# Autodesk Inventor assembly: Tiger
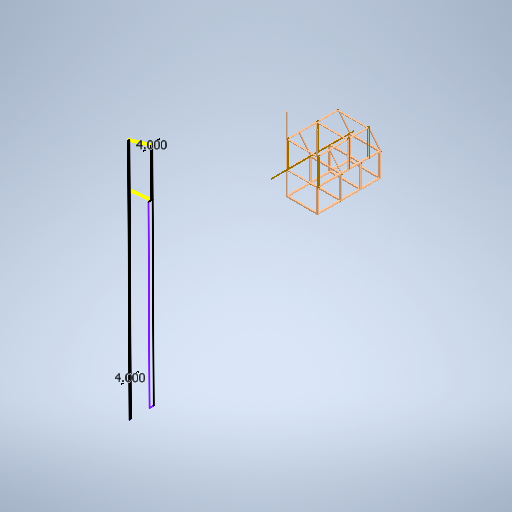
[picture p0: Inventor's stored thumbnail of the model, 512x512]
Saved by Autodesk Inventor 2025 (Build 290162000, 162)
## iProperties
Created: 2024-06-05
Part Number: Tiger
Document SubType Name: Assembly
Designer: Cupri
Mass: 180546 g
Surface Area: 136258 cm^2
Volume: 328266 cm^3
Density: 0.55 g/cm^3
Author: Cupri
## Documents named in this file (44)
- C:\Users\Win\Documents\GitHub\USCTigerBurn24\v2\Tiger.iam
- C:\Users\Win\Documents\GitHub\USCTigerBurn24\Standard Timber\4x4x72.ipt
- C:\Users\Win\Documents\GitHub\USCTigerBurn24\Standard Timber\4x4x40.ipt
- C:\Users\Win\Documents\GitHub\USCTigerBurn24\Standard Timber\2x4x36.ipt
- C:\Users\Win\Documents\GitHub\USCTigerBurn24\Standard Timber\2x4x40.ipt
- C:\Users\Win\Documents\GitHub\USCTigerBurn24\Standard Timber\2x4x24.ipt
- C:\Users\Win\Documents\GitHub\USCTigerBurn24\Standard Timber\2x4x28.ipt
- C:\Users\Win\Documents\GitHub\USCTigerBurn24\Standard Timber\2x4x72 (45 90).ipt
- C:\Users\Win\Documents\GitHub\USCTigerBurn24\Standard Timber\2x4x68 (45 90).ipt
- C:\Users\Win\Documents\GitHub\USCTigerBurn24\Standard Timber\2x4x42.343 (45 90).ipt
- C:\Users\Win\Documents\GitHub\USCTigerBurn24\Standard Timber\2x4x72 (30 90).ipt
- C:\Users\Win\Documents\GitHub\USCTigerBurn24\Standard Timber\2x4x44.ipt
- C:\Users\Win\Documents\GitHub\USCTigerBurn24\Standard Timber\4x4x104.303.ipt
- C:\Users\Win\Documents\GitHub\USCTigerBurn24\Standard Timber\4x4xigiveup.ipt
- C:\Users\Win\Documents\GitHub\USCTigerBurn24\Standard Timber\4x4x96.ipt
- C:\Users\Win\Documents\GitHub\USCTigerBurn24\Standard Timber\2x4x96.ipt
- C:\Users\Win\Documents\GitHub\USCTigerBurn24\Standard Timber\2x4xidk.ipt
- C:\Users\Win\Documents\GitHub\USCTigerBurn24\Standard Timber\2x4x120.ipt
- C:\Users\Win\Documents\GitHub\USCTigerBurn24\Standard Timber\2x4x72.ipt
- C:\Users\Win\Documents\GitHub\USCTigerBurn24\Standard Timber\2x4x88.ipt
- C:\Users\Win\Documents\GitHub\USCTigerBurn24\Standard Timber\4x4x55.ipt
- C:\Users\Win\Documents\GitHub\USCTigerBurn24\Standard Timber\4x4x66.ipt
- C:\Users\Win\Documents\GitHub\USCTigerBurn24\Standard Timber\2x4x48.ipt
- C:\Users\Win\Documents\GitHub\USCTigerBurn24\Standard Timber\leg slant.ipt
- C:\Users\Win\Documents\GitHub\USCTigerBurn24\Standard Timber\Leg slant.2.ipt
- C:\Users\Win\Documents\GitHub\USCTigerBurn24\Standard Timber\2x4x48_MIR.ipt
- C:\Users\Win\Documents\GitHub\USCTigerBurn24\Standard Timber\2x4x72_MIR.ipt
- C:\Users\Win\Documents\GitHub\USCTigerBurn24\Standard Timber\2x4x36_MIR.ipt
- C:\Users\Win\Documents\GitHub\USCTigerBurn24\Standard Timber\2x4x24_MIR.ipt
- C:\Users\Win\Documents\GitHub\USCTigerBurn24\Standard Timber\2x4x28_MIR.ipt
- C:\Users\Win\Documents\GitHub\USCTigerBurn24\Standard Timber\leg slant_MIR.ipt
- C:\Users\Win\Documents\GitHub\USCTigerBurn24\Standard Timber\Leg slant.2_MIR.ipt
- C:\Users\Win\Documents\GitHub\USCTigerBurn24\Standard Timber\back slant.ipt
- C:\Users\Win\Documents\2x4x76.ipt
- C:\Users\Win\Documents\2X4X65.191.ipt
- C:\Users\Win\Documents\2X4X92.ipt
- C:\Users\Win\Documents\wrapping paper.ipt
- C:\Users\Win\Documents\paperbodyfront.ipt
- C:\Users\Win\Documents\GitHub\USCTigerBurn24\v2\Tiger\AIP\FEA\epzzwi8io.fins
- C:\Users\Win\Documents\GitHub\USCTigerBurn24\v2\Tiger\AIP\FEA\epzzwi8io.fsat
- C:\Users\Win\Documents\GitHub\USCTigerBurn24\v2\Tiger\AIP\FEA\epzzwi8io.ftes
- C:\Users\Win\Documents\GitHub\USCTigerBurn24\v2\Tiger\AIP\FEA\epzzwi8io.fwiz
- C:\Users\Win\Documents\GitHub\USCTigerBurn24\v2\Tiger\AIP\FEA\epzzwi8jk.fmsh
- C:\Users\Win\Documents\GitHub\USCTigerBurn24\v2\Tiger\AIP\FEA\epzzwi8jl.fres
## Components (212 placed, 37 different names)
1. 4x4x104.303:1 — Flush:221, Flush:222
2. 4x4x104.303:2 — Flush:221, Flush:222
3. 4x4xigiveup:1 — Mate:186
4. 4x4xigiveup:2 — Flush:237, Mate:187, Mate:188
5. 4x4x96:1 — Flush:232
6. 4x4x96:2 — Flush:232
7. 4x4x96:3 — Flush:230
8. 4x4x96:4 — Flush:230
9. 4x4x96:5
10. 2x4x96:1 — Mate:186, Flush:237, Mate:187, Mate:188, Mate:191
11. 2x4xidk:1 — Mate:189, Mate:190, Mate:191, Flush:241
12. 2x4xidk:2 — Mate:192, Flush:240, Flush:241
13. 4x4x66:3 — Mate:391, Flush:531, Flush:532, Mate:401
14. 4x4x66:4 — Mate:392, Flush:533, Flush:534, Flush:548, Mate:402
15. 4x4x66:5 — Mate:393, Flush:535, Flush:536, Flush:606
16. 4x4x66:6 — Flush:537, Mate:394, Flush:538
17. 4x4x66:7 — Mate:395, Flush:539, Flush:540, Mate:403
18. 4x4x66:8 — Mate:396, Flush:541, Flush:542, Flush:563
19. 4x4x66:9 — Mate:397, Flush:543, Flush:544
20. 4x4x66:10 — Mate:398, Flush:545, Flush:546, Mate:399, Flush:547
21. 2x4x120:6 — Flush:561, Flush:565, Flush:566, Flush:567, Mate:419, Flush:572, Mate:431, Flush:584
22. 2x4x120:7 — Flush:563, Flush:564, Mate:415, Mate:416, Flush:568, Mate:417, Mate:433, Flush:585
23. 2x4x72:11 — Mate:414, Flush:571, Mate:430, Flush:582, Flush:583
24. 2x4x72:12 — Flush:580, Flush:581, Mate:429
25. 2x4x88:5 — Mate:413, Flush:562
26. 2x4x88:6 — Flush:569
27. 2x4x88:7 — Flush:570, Mate:418, Mate:420, Flush:606
28. back slant:1 — Flush:565, Flush:566, Flush:567, Mate:437, Mate:438, Flush:588
29. back slant:2 — Mate:415, Mate:416, Flush:568, Mate:435, Mate:436, Flush:586
30. back slant:3 — Mate:417, Flush:571, Mate:418
31. back slant:4 — Mate:419, Flush:572, Mate:420, Flush:598, Flush:599
32. 2x4x76:5 — Flush:580, Flush:581, Mate:429, Mate:432, Flush:589, Flush:590, Flush:607
33. 2x4x76:6 — Mate:430, Flush:582, Flush:583, Mate:434, Flush:591, Mate:439, Flush:592
34. 2X4X65.191:3 — Mate:435, Mate:436, Flush:586, Flush:587, Mate:442, Flush:597, Mate:443
35. 2X4X65.191:4 — Mate:437, Mate:438, Flush:588, Flush:595
36. 2x4x76:7 — Mate:431, Flush:584, Mate:432, Flush:596
37. 2x4x76:8 — Mate:433, Flush:585, Mate:434, Flush:587
38. 2X4X92:1 — Flush:589, Flush:590, Mate:440, Flush:593, Flush:594, Mate:441, Mate:444, Flush:602, Flush:603, Flush:607
39. 2X4X92:2 — Flush:591, Mate:439, Flush:592, Mate:445, Flush:604, Flush:605
40. 2x4x88:9 — Mate:440, Flush:593, Flush:594, Flush:600
41. 2x4x88:10 — Mate:441, Flush:595, Flush:596
42. 2X4X92:3 — Mate:442, Flush:597, Mate:443
43. wrapping paper:1 — Flush:598, Flush:599
44. paperbodyfront:1 — Flush:600, Flush:601
45. 2x4x72:13 — Mate:445, Flush:604, Flush:605
46. 2x4x72:15 — Mate:444, Flush:602, Flush:603
47. 2x4x72 (45 90):1 — Flush:88
48. 2x4x68 (45 90):1 — Flush:44, Flush:88
49. 2x4x72 (45 90):2 — Flush:48, Mate:48, Flush:51, Mate:49
50. 2x4x72 (45 90):3 — Flush:44, Mate:45, Mate:50, Flush:52, Mate:51
51. 2x4x42.343 (45 90):1 — Flush:48
52. 2x4x42.343 (45 90):2 — Mate:45
53. 2x4x72 (30 90):1 — Mate:48, Flush:51, Mate:49, Flush:70, Flush:238, Mate:192, Flush:240
54. 2x4x72 (30 90):2 — Mate:50, Flush:52, Mate:51, Flush:71, Flush:72
55. 2x4x72 (45 90):4 — Mate:61, Flush:61, Flush:62
56. 2x4x68 (45 90):2 — Mate:61, Flush:61, Flush:62
57. 2x4x72 (45 90):5 — Flush:59, Mate:59, Mate:65, Flush:67, Flush:68
58. 2x4x72 (45 90):6 — Flush:63, Flush:64, Mate:68, Flush:73
59. 2x4x42.343 (45 90):3 — Flush:59, Mate:59
60. 2x4x42.343 (45 90):4 — Flush:63
61. 2x4x72 (30 90):3 — Mate:66, Flush:69, Flush:204, Mate:189
62. 2x4x72 (30 90):4 — Flush:64, Mate:67, Mate:69, Flush:239
63. 2x4x44:1 — Mate:67, Flush:71, Flush:72, Flush:239, Mate:190
64. 2x4x44:2 — Mate:65, Flush:67, Flush:68
65. 2x4x44:3 — Mate:66, Flush:69, Flush:70, Flush:204, Flush:238
66. 2x4x44:4 — Mate:68, Flush:73, Mate:69
67. 4x4x72:65
68. 4x4x72:66
69. 4x4x40:117
70. 4x4x40:118
71. 4x4x40:119
72. 4x4x40:120
73. 4x4x40:121
74. 4x4x40:122
75. 4x4x40:123
76. 4x4x40:124
77. 4x4x72:67
78. 4x4x72:68
79. 4x4x40:125
80. 4x4x40:126
81. 4x4x40:127
82. 2x4x40:7
83. 2x4x36:25
84. 2x4x36:26
85. 2x4x36:27
86. 2x4x36:28
87. 2x4x24:13
88. 2x4x24:14
89. 2x4x28:13
90. 2x4x28:14
91. 4x4x72:69
92. 4x4x72:70
93. 4x4x40:128
94. 4x4x40:129
95. 4x4x40:130
96. 4x4x40:131
97. 4x4x72:71
98. 4x4x72:72
99. 4x4x72:73
100. 4x4x72:74
101. 4x4x40:132
102. 4x4x40:133
103. 4x4x40:134
104. 4x4x40:135
105. 4x4x40:136
106. 4x4x40:137
107. 4x4x40:138
108. 4x4x40:139
109. 4x4x72:75
110. 4x4x72:76
111. 4x4x40:140
112. 4x4x40:141
113. 4x4x40:142
114. 2x4x40:8
115. 2x4x36:29
116. 2x4x36:30
117. 2x4x36:31
118. 2x4x36:32
119. 2x4x24:15
120. 2x4x24:16
121. 2x4x28:15
122. 2x4x28:16
123. 4x4x72:77
124. 4x4x72:78
125. 4x4x40:143
126. 4x4x40:144
127. 4x4x40:145
128. 4x4x40:146
129. 4x4x72:79
130. 4x4x72:80
131. 4x4x96:7 — Flush:393, Mate:316, Flush:405, Mate:318, Mate:393, Flush:535, Flush:536, Mate:398, Flush:545, Flush:546
132. 4x4x96:10 — Flush:396, Mate:314, Flush:397, Flush:399, Mate:395, Flush:539, Flush:540, Mate:396, Flush:541, Flush:542
133. 2x4x120:4 — Mate:303, Flush:371, Flush:372, Flush:385, Mate:310, Flush:386, Flush:387, Mate:311, Flush:389, Mate:312, Mate:403, Flush:561
134. 2x4x120:5 — Mate:302, Flush:369, Flush:370, Mate:414, Flush:564
135. 2x4x72:1 — Mate:302, Flush:369, Flush:370, Mate:399, Flush:547, Flush:548, Mate:400, Mate:402
136. 2x4x72:2 — Mate:303, Flush:371, Flush:372, Flush:391, Mate:313, Flush:549, Mate:401
137. 4x4x96:13 — Flush:403, Flush:404, Flush:406, Mate:317, Mate:391, Flush:531, Flush:532, Mate:392, Flush:533, Flush:534
138. 4x4x96:16 — Flush:394, Flush:395, Mate:315, Flush:400, Flush:401, Flush:537, Mate:394, Flush:538, Mate:397, Flush:543, Flush:544
139. 2x4x88:1 — Flush:385, Mate:310, Flush:386, Mate:413, Flush:562
140. 2x4x88:2 — Flush:387, Mate:311, Flush:569
141. 2x4x88:3 — Flush:389, Mate:312, Flush:570, Flush:601
142. 2x4x88:4 — Flush:391, Mate:313, Mate:400, Flush:549
143. 4x4x55:1 — Flush:393, Flush:394, Flush:395
144. 4x4x55:2 — Flush:396, Mate:314, Flush:397, Flush:527
145. 4x4x55:3 — Flush:399, Mate:315, Flush:530
146. 4x4x55:4 — Flush:400, Mate:316, Flush:401, Mate:389
147. 4x4x66:1 — Flush:403, Flush:404, Mate:318
148. 4x4x66:2 — Flush:405, Flush:406, Mate:317
149. 2x4x48:1 — Mate:319, Flush:407, Flush:408, Mate:322, Mate:330, Flush:422, Flush:423
150. 2x4x48:2 — Flush:409, Mate:320, Flush:410, Mate:321, Flush:411, Mate:328, Flush:419, Flush:461, Mate:347, Flush:527
151. 2x4x48:3 — Mate:319, Flush:407, Flush:408, Flush:409, Mate:320, Flush:410, Mate:327, Flush:417, Flush:418
152. 2x4x48:4 — Mate:321, Flush:411, Mate:322, Mate:329, Flush:420, Flush:421
153. 2x4x48:5 — Flush:452
154. 2x4x48:6 — Flush:426, Flush:427
155. 2x4x48:7 — Mate:331, Flush:424, Flush:425, Flush:430, Flush:431, Flush:453, Mate:339
156. 2x4x48:8 — Flush:428, Flush:429
157. 2x4x72:3 — Mate:327, Flush:417, Flush:418, Mate:331, Flush:424, Flush:425, Flush:430, Flush:431
158. 2x4x72:4 — Mate:328, Flush:419, Flush:426, Flush:427, Mate:346, Flush:462
159. 2x4x72:5 — Mate:329, Flush:420, Flush:421, Flush:428, Flush:429, Flush:464
160. 2x4x72:6 — Mate:330, Flush:422, Flush:423
161. 2x4x48:9 — Flush:445, Flush:446
162. 2x4x48:10 — Mate:337, Flush:449, Flush:450
163. 2x4x48:11
164. 2x4x48:12 — Flush:447, Flush:448, Mate:338, Mate:349, Flush:465, Flush:466
165. 2x4x72:7 — Flush:452, Flush:453, Mate:339
166. 2x4x72:8 — Mate:337, Flush:449, Flush:450
167. 2x4x72:9 — Flush:447, Flush:448, Flush:451, Mate:338
168. 2x4x72:10 — Flush:445, Flush:446, Flush:451
169. 2x4x36:33
170. 2x4x36:34 — Flush:463, Flush:464
171. 2x4x36:35 — Mate:348, Mate:390
172. 2x4x36:36 — Flush:461, Mate:347
173. 2x4x24:17
174. 2x4x24:18 — Mate:390
175. 2x4x28:17
176. 2x4x28:18
177. 2x4x48:13 — Mate:346, Flush:462, Mate:348, Flush:463
178. 2x4x48:14 — Mate:349, Flush:465, Flush:466, Flush:467, Flush:468, Flush:469, Flush:470
179. leg slant:1 — Flush:467, Flush:468
180. Leg slant.2:1 — Flush:469, Flush:470
181. 2x4x48_MIR:1 — Flush:473, Flush:474, Mate:351, Mate:352, Flush:494, Flush:495, Mate:362
182. 2x4x48_MIR:2 — Flush:471, Mate:350, Flush:472, Flush:475, Mate:353, Flush:489, Mate:360, Mate:371, Flush:519
183. 2x4x48_MIR:3 — Flush:471, Mate:350, Flush:472, Flush:473, Flush:474, Mate:351, Flush:485, Flush:486, Mate:359
184. 2x4x48_MIR:4 — Mate:352, Flush:475, Mate:353, Flush:492, Flush:493, Mate:361, Flush:530
185. 2x4x48_MIR:5 — Flush:477, Flush:479, Mate:355, Mate:356, Flush:502
186. 2x4x48_MIR:6 — Mate:354, Flush:476, Flush:478, Flush:480, Mate:357, Flush:487, Flush:488
187. 2x4x48_MIR:7 — Mate:354, Flush:476, Flush:477, Flush:478, Flush:479, Mate:355, Flush:481, Flush:482, Flush:483, Flush:484, Mate:358, Mate:367, Flush:501
188. 2x4x48_MIR:8 — Mate:356, Flush:480, Mate:357, Flush:490, Flush:491
189. 2x4x72_MIR:1 — Flush:481, Flush:482, Flush:483, Flush:484, Mate:358, Flush:485, Flush:486, Mate:359
190. 2x4x72_MIR:2 — Flush:487, Flush:488, Flush:489, Mate:360, Flush:524, Mate:377
191. 2x4x72_MIR:3 — Flush:490, Flush:491, Flush:492, Flush:493, Mate:361, Flush:518, Mate:389
192. 2x4x72_MIR:4 — Flush:494, Flush:495, Mate:362
193. 2x4x48_MIR:9 — Flush:497, Flush:499, Mate:364, Mate:365, Flush:516, Flush:517, Mate:385, Mate:404
194. 2x4x48_MIR:10 — Mate:363, Flush:496, Flush:498, Flush:500, Mate:366, Flush:507, Flush:508, Mate:369, Flush:509, Flush:510, Flush:529, Mate:387
195. 2x4x48_MIR:11 — Mate:363, Flush:496, Flush:497, Flush:498, Flush:499, Mate:364, Flush:503, Flush:504, Flush:505, Mate:368, Flush:506
196. 2x4x48_MIR:12 — Mate:365, Flush:500, Mate:366, Mate:370, Flush:511, Flush:512, Flush:513, Flush:514, Flush:525, Flush:526, Mate:378
197. 2x4x72_MIR:5 — Mate:367, Flush:501, Flush:502, Flush:503, Flush:504, Flush:505, Mate:368, Flush:506
198. 2x4x72_MIR:6 — Flush:507, Flush:508, Mate:369, Flush:509, Flush:510
199. 2x4x72_MIR:7 — Mate:370, Flush:511, Flush:512, Flush:513, Flush:514, Flush:515
200. 2x4x72_MIR:8 — Flush:515, Flush:516, Flush:517
201. 2x4x36_MIR:1 — Flush:522, Mate:375, Rigid:233
202. 2x4x36_MIR:2 — Flush:518, Mate:373, Flush:520, Mate:374, Flush:521, Flush:523
203. 2x4x36_MIR:3 — Mate:372, Mate:376, Rigid:235, Mate:388
204. 2x4x36_MIR:4 — Mate:371, Flush:519, Mate:372, Rigid:234, Rigid:236
205. 2x4x24_MIR:1 — Mate:373, Flush:520, Rigid:233
206. 2x4x24_MIR:2 — Rigid:234, Mate:388
207. 2x4x28_MIR:1 — Mate:374, Flush:521, Rigid:235
208. 2x4x28_MIR:2 — Flush:522, Mate:375, Rigid:236
209. 2x4x48_MIR:13 — Flush:523, Mate:376, Flush:524, Mate:377
210. 2x4x48_MIR:14 — Flush:525, Flush:526, Mate:378, Mate:379, Mate:380, Mate:381, Mate:382, Mate:384, Mate:386, Flush:550, Mate:405
211. leg slant_MIR:1 — Mate:379, Mate:380, Mate:384, Mate:385, Mate:404, Flush:550, Mate:405
212. Leg slant.2_MIR:1 — Mate:381, Mate:382, Mate:386, Flush:529, Mate:387
## Relationships (498: Flush 276, Mate 176, WeldJoint 46)
- Flush:44: 2x4x68 (45 90):1 ↔ 2x4x72 (45 90):3
- Flush:48: 2x4x72 (45 90):2 ↔ 2x4x42.343 (45 90):1
- Mate:45: 2x4x72 (45 90):3 ↔ 2x4x42.343 (45 90):2
- Mate:48: 2x4x72 (45 90):2 ↔ 2x4x72 (30 90):1
- Flush:51: 2x4x72 (45 90):2 ↔ 2x4x72 (30 90):1
- Mate:49: 2x4x72 (45 90):2 ↔ 2x4x72 (30 90):1
- Mate:50: 2x4x72 (45 90):3 ↔ 2x4x72 (30 90):2
- Flush:52: 2x4x72 (45 90):3 ↔ 2x4x72 (30 90):2
- Mate:51: 2x4x72 (45 90):3 ↔ 2x4x72 (30 90):2
- [Flush]: 2x4x68 (45 90):2 ↔ 2x4x72 (45 90):6
- [Flush]: 2x4x72 (45 90):5 ↔ 2x4x42.343 (45 90):3
- [Mate]: 2x4x72 (45 90):6 ↔ 2x4x42.343 (45 90):4
- [Mate]: 2x4x72 (45 90):5 ↔ 2x4x72 (30 90):3
- [Flush]: 2x4x72 (45 90):5 ↔ 2x4x72 (30 90):3
- [Mate]: 2x4x72 (45 90):5 ↔ 2x4x72 (30 90):3
- [Mate]: 2x4x72 (45 90):6 ↔ 2x4x72 (30 90):4
- [Flush]: 2x4x72 (45 90):6 ↔ 2x4x72 (30 90):4
- [Mate]: 2x4x72 (45 90):6 ↔ 2x4x72 (30 90):4
- Flush:59: 2x4x72 (45 90):5 ↔ 2x4x42.343 (45 90):3
- Mate:59: 2x4x72 (45 90):5 ↔ 2x4x42.343 (45 90):3
- Mate:61: 2x4x72 (45 90):4 ↔ 2x4x68 (45 90):2
- Flush:61: 2x4x72 (45 90):4 ↔ 2x4x68 (45 90):2
- Flush:62: 2x4x72 (45 90):4 ↔ 2x4x68 (45 90):2
- Flush:63: 2x4x72 (45 90):6 ↔ 2x4x42.343 (45 90):4
- Flush:64: 2x4x72 (45 90):6 ↔ 2x4x72 (30 90):4
- Mate:65: 2x4x72 (45 90):5 ↔ 2x4x44:2
- Flush:67: 2x4x72 (45 90):5 ↔ 2x4x44:2
- Flush:68: 2x4x72 (45 90):5 ↔ 2x4x44:2
- Mate:66: 2x4x72 (30 90):3 ↔ 2x4x44:3
- Flush:69: 2x4x72 (30 90):3 ↔ 2x4x44:3
- Flush:70: 2x4x72 (30 90):1 ↔ 2x4x44:3
- Mate:67: 2x4x72 (30 90):4 ↔ 2x4x44:1
- Flush:71: 2x4x72 (30 90):2 ↔ 2x4x44:1
- Flush:72: 2x4x72 (30 90):2 ↔ 2x4x44:1
- Mate:68: 2x4x72 (45 90):6 ↔ 2x4x44:4
- Flush:73: 2x4x72 (45 90):6 ↔ 2x4x44:4
- Mate:69: 2x4x72 (30 90):4 ↔ 2x4x44:4
- Flush:88: 2x4x72 (45 90):1 ↔ 2x4x68 (45 90):1
- Flush:204: 2x4x72 (30 90):3 ↔ 2x4x44:3
- Flush:221: 4x4x104.303:1 ↔ 4x4x104.303:2
- Flush:222: 4x4x104.303:1 ↔ 4x4x104.303:2
- Flush:230: 4x4x96:3 ↔ 4x4x96:4
- Flush:232: 4x4x96:1 ↔ 4x4x96:2
- Mate:186: 4x4xigiveup:1 ↔ 2x4x96:1
- Flush:237: 4x4xigiveup:2 ↔ 2x4x96:1
- Mate:187: 4x4xigiveup:2 ↔ 2x4x96:1
- Mate:188: 4x4xigiveup:2 ↔ 2x4x96:1
- Flush:238: 2x4x72 (30 90):1 ↔ 2x4x44:3
- Flush:239: 2x4x72 (30 90):4 ↔ 2x4x44:1
- Mate:189: 2x4xidk:1 ↔ 2x4x72 (30 90):3
- Mate:190: 2x4xidk:1 ↔ 2x4x44:1
- Mate:191: 2x4x96:1 ↔ 2x4xidk:1
- Mate:192: 2x4xidk:2 ↔ 2x4x72 (30 90):1
- Flush:240: 2x4xidk:2 ↔ 2x4x72 (30 90):1
- Flush:241: 2x4xidk:1 ↔ 2x4xidk:2
- [WeldJoint]: 4x4x72:65 ↔ 4x4x40:117
- [WeldJoint]: 4x4x72:66 ↔ 4x4x40:117
- [WeldJoint]: 4x4x72:65 ↔ 4x4x40:118
- [WeldJoint]: 4x4x72:66 ↔ 4x4x40:120
- [WeldJoint]: 4x4x40:118 ↔ 4x4x72:67
- [WeldJoint]: 4x4x40:119 ↔ 4x4x72:67
- [WeldJoint]: 4x4x40:120 ↔ 4x4x72:68
- [WeldJoint]: 4x4x72:66 ↔ 4x4x40:121
- [WeldJoint]: 4x4x40:122 ↔ 4x4x72:67
- [WeldJoint]: 4x4x72:65 ↔ 4x4x40:124
- [WeldJoint]: 4x4x72:65 ↔ 4x4x40:123
- [Mate]: 4x4x72:67 ↔ 2x4x40:7
- [Flush]: 4x4x72:67 ↔ 2x4x40:7
- [Mate] (609.6 mm): 4x4x40:119 ↔ 2x4x40:7
- [Mate] (101.6 mm): 4x4x40:119 ↔ 2x4x36:25
- [Flush]: 4x4x40:119 ↔ 2x4x36:25
- [Mate] (101.6 mm): 4x4x72:68 ↔ 2x4x36:28
- [Flush]: 4x4x40:119 ↔ 2x4x36:28
- [Mate] (101.6 mm): 2x4x40:7 ↔ 2x4x36:26
- [Flush]: 2x4x40:7 ↔ 2x4x36:26
- [Mate]: 2x4x40:7 ↔ 2x4x36:27
- [Flush]: 2x4x40:7 ↔ 2x4x36:27
- [Mate]: 2x4x36:27 ↔ 2x4x36:28
- [WeldJoint]: 2x4x36:25 ↔ 2x4x24:13
- [WeldJoint]: 2x4x36:28 ↔ 2x4x24:14
- [WeldJoint]: 2x4x36:27 ↔ 2x4x28:13
- [WeldJoint]: 2x4x36:28 ↔ 2x4x28:14
- [WeldJoint]: 4x4x72:70 ↔ 4x4x40:128
- [WeldJoint]: 4x4x40:129 ↔ 4x4x72:71
- [WeldJoint]: 4x4x72:69 ↔ 4x4x40:131
- [WeldJoint]: 4x4x72:69 ↔ 4x4x40:130
- [Flush]: 2x4x40:7 ↔ 2x4x36:26
- [Flush]: 2x4x40:7 ↔ 2x4x36:27
- [Flush]: 4x4x40:119 ↔ 2x4x36:25
- [Flush]: 4x4x40:119 ↔ 2x4x36:28
- [Flush] (203.2 mm): 4x4x72:68 ↔ 2x4x36:27
- [Flush] (203.2 mm): 4x4x72:68 ↔ 2x4x36:28
- [Flush]: 2x4x36:25 ↔ 2x4x28:14
- [Mate]: 2x4x36:26 ↔ 2x4x28:13
- [Flush]: 4x4x40:129 ↔ 4x4x72:71
- [Flush]: 4x4x40:129 ↔ 4x4x72:72
- [Mate]: 4x4x40:129 ↔ 4x4x72:72
- [Mate]: 4x4x40:128 ↔ 4x4x72:72
- [Flush]: 4x4x40:128 ↔ 4x4x72:72
- [Flush]: 4x4x72:70 ↔ 4x4x40:128
- [Mate]: 4x4x72:70 ↔ 4x4x40:128
- [Flush]: 4x4x72:69 ↔ 4x4x40:131
- [Flush]: 4x4x72:69 ↔ 4x4x40:130
- [Mate]: 4x4x72:67 ↔ 2x4x40:7
- [Mate]: 2x4x36:26 ↔ 2x4x24:13
- [Flush]: 4x4x72:68 ↔ 4x4x72:72
- [Flush]: 4x4x72:68 ↔ 4x4x72:72
- [WeldJoint]: 4x4x72:73 ↔ 4x4x40:132
- [WeldJoint]: 4x4x72:74 ↔ 4x4x40:132
- [WeldJoint]: 4x4x72:73 ↔ 4x4x40:133
- [WeldJoint]: 4x4x72:74 ↔ 4x4x40:135
- [WeldJoint]: 4x4x40:133 ↔ 4x4x72:75
- [WeldJoint]: 4x4x40:134 ↔ 4x4x72:75
- [WeldJoint]: 4x4x40:135 ↔ 4x4x72:76
- [WeldJoint]: 4x4x72:74 ↔ 4x4x40:136
- [WeldJoint]: 4x4x40:137 ↔ 4x4x72:75
- [WeldJoint]: 4x4x72:73 ↔ 4x4x40:139
- [WeldJoint]: 4x4x72:73 ↔ 4x4x40:138
- [Mate]: 4x4x72:75 ↔ 2x4x40:8
- [Flush]: 4x4x72:75 ↔ 2x4x40:8
- [Mate] (609.6 mm): 4x4x40:134 ↔ 2x4x40:8
- [Mate] (101.6 mm): 4x4x40:134 ↔ 2x4x36:29
- [Flush]: 4x4x40:134 ↔ 2x4x36:29
- [Mate] (101.6 mm): 4x4x72:76 ↔ 2x4x36:32
- [Flush]: 4x4x40:134 ↔ 2x4x36:32
- [Mate]: 2x4x40:8 ↔ 2x4x36:31
- [Flush]: 2x4x40:8 ↔ 2x4x36:31
- [Mate]: 2x4x36:31 ↔ 2x4x36:32
- [WeldJoint]: 2x4x36:29 ↔ 2x4x24:15
- [WeldJoint]: 2x4x36:32 ↔ 2x4x24:16
- [WeldJoint]: 2x4x36:31 ↔ 2x4x28:15
- [WeldJoint]: 2x4x36:32 ↔ 2x4x28:16
- [WeldJoint]: 4x4x72:78 ↔ 4x4x40:143
- [WeldJoint]: 4x4x40:144 ↔ 4x4x72:79
- [WeldJoint]: 4x4x72:77 ↔ 4x4x40:146
- [WeldJoint]: 4x4x72:77 ↔ 4x4x40:145
- [Flush]: 2x4x40:8 ↔ 2x4x36:31
- [Flush]: 4x4x40:134 ↔ 2x4x36:29
- [Flush]: 4x4x40:134 ↔ 2x4x36:32
- [Flush] (203.2 mm): 4x4x72:76 ↔ 2x4x36:31
- [Flush] (203.2 mm): 4x4x72:76 ↔ 2x4x36:32
- [Flush]: 2x4x36:29 ↔ 2x4x28:16
- [Flush]: 2x4x36:30 ↔ 2x4x28:15
- [Mate]: 2x4x36:30 ↔ 2x4x28:15
- [Flush]: 4x4x40:144 ↔ 4x4x72:79
- [Flush]: 4x4x40:144 ↔ 4x4x72:80
- [Mate]: 4x4x40:144 ↔ 4x4x72:79
- [Mate]: 4x4x40:146 ↔ 4x4x72:79
- [Mate]: 4x4x72:74 ↔ 4x4x72:78
- [Mate]: 4x4x72:75 ↔ 2x4x40:8
- [Mate]: 2x4x40:8 ↔ 2x4x24:15
- [Flush]: 2x4x36:31 ↔ 2x4x24:16
- [Flush]: 2x4x36:31 ↔ 2x4x24:16
- [Mate]: 2x4x40:8 ↔ 2x4x36:30
- [Flush]: 2x4x36:30 ↔ 2x4x28:15
- [Flush]: 2x4x36:30 ↔ 2x4x28:15
- [Mate]: 4x4x72:78 ↔ 4x4x40:145
- Mate:302: 2x4x120:5 ↔ 2x4x72:1
- Flush:369: 2x4x120:5 ↔ 2x4x72:1
- Flush:370: 2x4x120:5 ↔ 2x4x72:1
- Mate:303: 2x4x120:4 ↔ 2x4x72:2
- Flush:371: 2x4x120:4 ↔ 2x4x72:2
- Flush:372: 2x4x120:4 ↔ 2x4x72:2
- Flush:385: 2x4x120:4 ↔ 2x4x88:1
- Mate:310: 2x4x120:4 ↔ 2x4x88:1
- Flush:386: 2x4x120:4 ↔ 2x4x88:1
- Flush:387: 2x4x120:4 ↔ 2x4x88:2
- Mate:311: 2x4x120:4 ↔ 2x4x88:2
- Flush:389: 2x4x120:4 ↔ 2x4x88:3
- Mate:312: 2x4x120:4 ↔ 2x4x88:3
- Flush:391: 2x4x72:2 ↔ 2x4x88:4
- Mate:313: 2x4x72:2 ↔ 2x4x88:4
- Flush:393: 4x4x96:7 ↔ 4x4x55:1
- Flush:394: 4x4x96:16 ↔ 4x4x55:1
- Flush:395: 4x4x96:16 ↔ 4x4x55:1
- Flush:396: 4x4x96:10 ↔ 4x4x55:2
- Mate:314: 4x4x96:10 ↔ 4x4x55:2
- Flush:397: 4x4x96:10 ↔ 4x4x55:2
- Flush:399: 4x4x96:10 ↔ 4x4x55:3
- Mate:315: 4x4x96:16 ↔ 4x4x55:3
- Flush:400: 4x4x96:16 ↔ 4x4x55:4
- Mate:316: 4x4x96:7 ↔ 4x4x55:4
- Flush:401: 4x4x96:16 ↔ 4x4x55:4
- Flush:403: 4x4x96:13 ↔ 4x4x66:1
- Flush:404: 4x4x96:13 ↔ 4x4x66:1
- Flush:405: 4x4x96:7 ↔ 4x4x66:2
- Flush:406: 4x4x96:13 ↔ 4x4x66:2
- Mate:317: 4x4x96:13 ↔ 4x4x66:2
- Mate:318: 4x4x96:7 ↔ 4x4x66:1
- Mate:319: 2x4x48:1 ↔ 2x4x48:3
- Flush:407: 2x4x48:1 ↔ 2x4x48:3
- Flush:408: 2x4x48:1 ↔ 2x4x48:3
- Flush:409: 2x4x48:2 ↔ 2x4x48:3
- Mate:320: 2x4x48:2 ↔ 2x4x48:3
- Flush:410: 2x4x48:2 ↔ 2x4x48:3
- Mate:321: 2x4x48:2 ↔ 2x4x48:4
- Flush:411: 2x4x48:2 ↔ 2x4x48:4
- Mate:322: 2x4x48:1 ↔ 2x4x48:4
- [Mate]: 2x4x48:5 ↔ 2x4x48:7
- [Flush]: 2x4x48:5 ↔ 2x4x48:7
- [Flush]: 2x4x48:5 ↔ 2x4x48:7
- [Flush]: 2x4x48:6 ↔ 2x4x48:7
- [Mate]: 2x4x48:6 ↔ 2x4x48:7
- [Flush]: 2x4x48:6 ↔ 2x4x48:7
- [Mate]: 2x4x48:6 ↔ 2x4x48:8
- [Flush]: 2x4x48:6 ↔ 2x4x48:8
- [Mate]: 2x4x48:5 ↔ 2x4x48:8
- Mate:327: 2x4x48:3 ↔ 2x4x72:3
- Flush:417: 2x4x48:3 ↔ 2x4x72:3
- Flush:418: 2x4x48:3 ↔ 2x4x72:3
- Mate:328: 2x4x48:2 ↔ 2x4x72:4
- Flush:419: 2x4x48:2 ↔ 2x4x72:4
- Mate:329: 2x4x48:4 ↔ 2x4x72:5
- Flush:420: 2x4x48:4 ↔ 2x4x72:5
- Flush:421: 2x4x48:4 ↔ 2x4x72:5
- Mate:330: 2x4x48:1 ↔ 2x4x72:6
- Flush:422: 2x4x48:1 ↔ 2x4x72:6
- Flush:423: 2x4x48:1 ↔ 2x4x72:6
- Mate:331: 2x4x48:7 ↔ 2x4x72:3
- Flush:424: 2x4x48:7 ↔ 2x4x72:3
- Flush:425: 2x4x48:7 ↔ 2x4x72:3
- Flush:426: 2x4x48:6 ↔ 2x4x72:4
- Flush:427: 2x4x48:6 ↔ 2x4x72:4
- Flush:428: 2x4x48:8 ↔ 2x4x72:5
- Flush:429: 2x4x48:8 ↔ 2x4x72:5
- Flush:430: 2x4x48:7 ↔ 2x4x72:3
- Flush:431: 2x4x48:7 ↔ 2x4x72:3
- [Mate]: 2x4x48:9 ↔ 2x4x48:11
- [Flush]: 2x4x48:9 ↔ 2x4x48:11
- [Flush]: 2x4x48:9 ↔ 2x4x48:11
- [Flush]: 2x4x48:10 ↔ 2x4x48:11
- [Mate]: 2x4x48:10 ↔ 2x4x48:11
- [Flush]: 2x4x48:10 ↔ 2x4x48:11
- [Mate]: 2x4x48:10 ↔ 2x4x48:12
- [Flush]: 2x4x48:10 ↔ 2x4x48:12
- [Mate]: 2x4x48:9 ↔ 2x4x48:12
- [Mate]: 2x4x48:11 ↔ 2x4x72:7
- [Flush]: 2x4x48:11 ↔ 2x4x72:7
- [Flush]: 2x4x48:11 ↔ 2x4x72:7
- [Flush]: 2x4x48:10 ↔ 2x4x72:8
- [Flush]: 2x4x48:10 ↔ 2x4x72:8
- [Flush]: 2x4x48:12 ↔ 2x4x72:9
- [Flush]: 2x4x48:12 ↔ 2x4x72:9
- [Flush]: 2x4x48:11 ↔ 2x4x72:7
- [Flush]: 2x4x48:11 ↔ 2x4x72:7
- Mate:337: 2x4x48:10 ↔ 2x4x72:8
- Flush:445: 2x4x48:9 ↔ 2x4x72:10
- Flush:446: 2x4x48:9 ↔ 2x4x72:10
- Flush:447: 2x4x48:12 ↔ 2x4x72:9
- Flush:448: 2x4x48:12 ↔ 2x4x72:9
- Flush:449: 2x4x48:10 ↔ 2x4x72:8
- Flush:450: 2x4x48:10 ↔ 2x4x72:8
- Flush:451: 2x4x72:9 ↔ 2x4x72:10
- Mate:338: 2x4x48:12 ↔ 2x4x72:9
- Flush:452: 2x4x48:5 ↔ 2x4x72:7
- Flush:453: 2x4x48:7 ↔ 2x4x72:7
- Mate:339: 2x4x48:7 ↔ 2x4x72:7
- [Mate]: 2x4x36:35 ↔ 2x4x36:36
- [WeldJoint]: 2x4x36:33 ↔ 2x4x24:17
- [WeldJoint]: 2x4x36:36 ↔ 2x4x24:18
- [WeldJoint]: 2x4x36:35 ↔ 2x4x28:17
- [WeldJoint]: 2x4x36:36 ↔ 2x4x28:18
- [Flush]: 2x4x36:33 ↔ 2x4x28:18
- [Mate]: 2x4x36:34 ↔ 2x4x28:17
- [Mate]: 2x4x36:34 ↔ 2x4x24:17
- [Mate]: 2x4x36:33 ↔ 2x4x28:18
- [Flush]: 2x4x36:34 ↔ 2x4x24:17
- [Flush]: 2x4x36:34 ↔ 2x4x28:17
- Flush:461: 2x4x48:2 ↔ 2x4x36:36
- Mate:346: 2x4x72:4 ↔ 2x4x48:13
- Flush:462: 2x4x72:4 ↔ 2x4x48:13
- Mate:347: 2x4x48:2 ↔ 2x4x36:36
- Mate:348: 2x4x36:35 ↔ 2x4x48:13
- Flush:463: 2x4x36:34 ↔ 2x4x48:13
- Flush:464 (254 mm): 2x4x72:5 ↔ 2x4x36:34
- Mate:349: 2x4x48:12 ↔ 2x4x48:14
- Flush:465: 2x4x48:12 ↔ 2x4x48:14
- Flush:466: 2x4x48:12 ↔ 2x4x48:14
- Flush:467: 2x4x48:14 ↔ leg slant:1
- Flush:468: 2x4x48:14 ↔ leg slant:1
- Flush:469: 2x4x48:14 ↔ Leg slant.2:1
- Flush:470: 2x4x48:14 ↔ Leg slant.2:1
- Flush:471: 2x4x48_MIR:2 ↔ 2x4x48_MIR:3
- Mate:350: 2x4x48_MIR:2 ↔ 2x4x48_MIR:3
- Flush:472: 2x4x48_MIR:2 ↔ 2x4x48_MIR:3
- Flush:473: 2x4x48_MIR:1 ↔ 2x4x48_MIR:3
- Flush:474: 2x4x48_MIR:1 ↔ 2x4x48_MIR:3
- Mate:351: 2x4x48_MIR:1 ↔ 2x4x48_MIR:3
- Mate:352: 2x4x48_MIR:1 ↔ 2x4x48_MIR:4
- Flush:475: 2x4x48_MIR:2 ↔ 2x4x48_MIR:4
- Mate:353: 2x4x48_MIR:2 ↔ 2x4x48_MIR:4
- Mate:354: 2x4x48_MIR:6 ↔ 2x4x48_MIR:7
- Flush:476: 2x4x48_MIR:6 ↔ 2x4x48_MIR:7
- Flush:477: 2x4x48_MIR:5 ↔ 2x4x48_MIR:7
- Flush:478: 2x4x48_MIR:6 ↔ 2x4x48_MIR:7
- Flush:479: 2x4x48_MIR:5 ↔ 2x4x48_MIR:7
- Mate:355: 2x4x48_MIR:5 ↔ 2x4x48_MIR:7
- Mate:356: 2x4x48_MIR:5 ↔ 2x4x48_MIR:8
- Flush:480: 2x4x48_MIR:6 ↔ 2x4x48_MIR:8
- Mate:357: 2x4x48_MIR:6 ↔ 2x4x48_MIR:8
- Flush:481: 2x4x48_MIR:7 ↔ 2x4x72_MIR:1
- Flush:482: 2x4x48_MIR:7 ↔ 2x4x72_MIR:1
- Flush:483: 2x4x48_MIR:7 ↔ 2x4x72_MIR:1
- Flush:484: 2x4x48_MIR:7 ↔ 2x4x72_MIR:1
- Mate:358: 2x4x48_MIR:7 ↔ 2x4x72_MIR:1
- Flush:485: 2x4x48_MIR:3 ↔ 2x4x72_MIR:1
- Flush:486: 2x4x48_MIR:3 ↔ 2x4x72_MIR:1
- Mate:359: 2x4x48_MIR:3 ↔ 2x4x72_MIR:1
- Flush:487: 2x4x48_MIR:6 ↔ 2x4x72_MIR:2
- Flush:488: 2x4x48_MIR:6 ↔ 2x4x72_MIR:2
- Flush:489: 2x4x48_MIR:2 ↔ 2x4x72_MIR:2
- Mate:360: 2x4x48_MIR:2 ↔ 2x4x72_MIR:2
- Flush:490: 2x4x48_MIR:8 ↔ 2x4x72_MIR:3
- Flush:491: 2x4x48_MIR:8 ↔ 2x4x72_MIR:3
- Flush:492: 2x4x48_MIR:4 ↔ 2x4x72_MIR:3
- Flush:493: 2x4x48_MIR:4 ↔ 2x4x72_MIR:3
- Mate:361: 2x4x48_MIR:4 ↔ 2x4x72_MIR:3
- Flush:494: 2x4x48_MIR:1 ↔ 2x4x72_MIR:4
- Flush:495: 2x4x48_MIR:1 ↔ 2x4x72_MIR:4
- Mate:362: 2x4x48_MIR:1 ↔ 2x4x72_MIR:4
- Mate:363: 2x4x48_MIR:10 ↔ 2x4x48_MIR:11
- Flush:496: 2x4x48_MIR:10 ↔ 2x4x48_MIR:11
- Flush:497: 2x4x48_MIR:9 ↔ 2x4x48_MIR:11
- Flush:498: 2x4x48_MIR:10 ↔ 2x4x48_MIR:11
- Flush:499: 2x4x48_MIR:9 ↔ 2x4x48_MIR:11
- Mate:364: 2x4x48_MIR:9 ↔ 2x4x48_MIR:11
- Mate:365: 2x4x48_MIR:9 ↔ 2x4x48_MIR:12
- Flush:500: 2x4x48_MIR:10 ↔ 2x4x48_MIR:12
- Mate:366: 2x4x48_MIR:10 ↔ 2x4x48_MIR:12
- Mate:367: 2x4x48_MIR:7 ↔ 2x4x72_MIR:5
- Flush:501: 2x4x48_MIR:7 ↔ 2x4x72_MIR:5
- Flush:502: 2x4x48_MIR:5 ↔ 2x4x72_MIR:5
- Flush:503: 2x4x48_MIR:11 ↔ 2x4x72_MIR:5
- Flush:504: 2x4x48_MIR:11 ↔ 2x4x72_MIR:5
- Flush:505: 2x4x48_MIR:11 ↔ 2x4x72_MIR:5
- Mate:368: 2x4x48_MIR:11 ↔ 2x4x72_MIR:5
- Flush:506: 2x4x48_MIR:11 ↔ 2x4x72_MIR:5
- Flush:507: 2x4x48_MIR:10 ↔ 2x4x72_MIR:6
- Flush:508: 2x4x48_MIR:10 ↔ 2x4x72_MIR:6
- Mate:369: 2x4x48_MIR:10 ↔ 2x4x72_MIR:6
- Flush:509: 2x4x48_MIR:10 ↔ 2x4x72_MIR:6
- Flush:510: 2x4x48_MIR:10 ↔ 2x4x72_MIR:6
- Mate:370: 2x4x48_MIR:12 ↔ 2x4x72_MIR:7
- Flush:511: 2x4x48_MIR:12 ↔ 2x4x72_MIR:7
- Flush:512: 2x4x48_MIR:12 ↔ 2x4x72_MIR:7
- Flush:513: 2x4x48_MIR:12 ↔ 2x4x72_MIR:7
- Flush:514: 2x4x48_MIR:12 ↔ 2x4x72_MIR:7
- Flush:515: 2x4x72_MIR:7 ↔ 2x4x72_MIR:8
- Flush:516: 2x4x48_MIR:9 ↔ 2x4x72_MIR:8
- Flush:517: 2x4x48_MIR:9 ↔ 2x4x72_MIR:8
- Flush:518 (254 mm): 2x4x72_MIR:3 ↔ 2x4x36_MIR:2
- Mate:371: 2x4x48_MIR:2 ↔ 2x4x36_MIR:4
- Flush:519: 2x4x48_MIR:2 ↔ 2x4x36_MIR:4
- Mate:372: 2x4x36_MIR:3 ↔ 2x4x36_MIR:4
- Mate:373: 2x4x36_MIR:2 ↔ 2x4x24_MIR:1
- Flush:520: 2x4x36_MIR:2 ↔ 2x4x24_MIR:1
- Mate:374: 2x4x36_MIR:2 ↔ 2x4x28_MIR:1
- Flush:521: 2x4x36_MIR:2 ↔ 2x4x28_MIR:1
- Flush:522: 2x4x36_MIR:1 ↔ 2x4x28_MIR:2
- Mate:375: 2x4x36_MIR:1 ↔ 2x4x28_MIR:2
- Flush:523: 2x4x36_MIR:2 ↔ 2x4x48_MIR:13
- Mate:376: 2x4x36_MIR:3 ↔ 2x4x48_MIR:13
- Flush:524: 2x4x72_MIR:2 ↔ 2x4x48_MIR:13
- Mate:377: 2x4x72_MIR:2 ↔ 2x4x48_MIR:13
- Flush:525: 2x4x48_MIR:12 ↔ 2x4x48_MIR:14
- Flush:526: 2x4x48_MIR:12 ↔ 2x4x48_MIR:14
- Mate:378: 2x4x48_MIR:12 ↔ 2x4x48_MIR:14
- Mate:379: 2x4x48_MIR:14 ↔ leg slant_MIR:1
- Mate:380: 2x4x48_MIR:14 ↔ leg slant_MIR:1
- Mate:381: 2x4x48_MIR:14 ↔ Leg slant.2_MIR:1
- Mate:382: 2x4x48_MIR:14 ↔ Leg slant.2_MIR:1
- Rigid:233 [WeldJoint]: 2x4x36_MIR:1 ↔ 2x4x24_MIR:1
- Rigid:234 [WeldJoint]: 2x4x36_MIR:4 ↔ 2x4x24_MIR:2
- Rigid:235 [WeldJoint]: 2x4x36_MIR:3 ↔ 2x4x28_MIR:1
- Rigid:236 [WeldJoint]: 2x4x36_MIR:4 ↔ 2x4x28_MIR:2
- Flush:527: 4x4x55:2 ↔ 2x4x48:2
- Mate:384: 2x4x48_MIR:14 ↔ leg slant_MIR:1
- Mate:385: 2x4x48_MIR:9 ↔ leg slant_MIR:1
- Mate:386: 2x4x48_MIR:14 ↔ Leg slant.2_MIR:1
- Flush:529: 2x4x48_MIR:10 ↔ Leg slant.2_MIR:1
- Mate:387: 2x4x48_MIR:10 ↔ Leg slant.2_MIR:1
- Mate:388: 2x4x36_MIR:3 ↔ 2x4x24_MIR:2
- Mate:389: 4x4x55:4 ↔ 2x4x72_MIR:3
- Flush:530: 4x4x55:3 ↔ 2x4x48_MIR:4
- Mate:390: 2x4x36:35 ↔ 2x4x24:18
- Mate:391: 4x4x66:3 ↔ 4x4x96:13
- Flush:531: 4x4x66:3 ↔ 4x4x96:13
- Flush:532: 4x4x66:3 ↔ 4x4x96:13
- Mate:392: 4x4x66:4 ↔ 4x4x96:13
- Flush:533: 4x4x66:4 ↔ 4x4x96:13
- Flush:534: 4x4x66:4 ↔ 4x4x96:13
- Mate:393: 4x4x66:5 ↔ 4x4x96:7
- Flush:535: 4x4x66:5 ↔ 4x4x96:7
- Flush:536: 4x4x66:5 ↔ 4x4x96:7
- Flush:537: 4x4x66:6 ↔ 4x4x96:16
- Mate:394: 4x4x66:6 ↔ 4x4x96:16
- Flush:538: 4x4x66:6 ↔ 4x4x96:16
- Mate:395: 4x4x66:7 ↔ 4x4x96:10
- Flush:539: 4x4x66:7 ↔ 4x4x96:10
- Flush:540: 4x4x66:7 ↔ 4x4x96:10
- Mate:396: 4x4x66:8 ↔ 4x4x96:10
- Flush:541: 4x4x66:8 ↔ 4x4x96:10
- Flush:542: 4x4x66:8 ↔ 4x4x96:10
- Mate:397: 4x4x66:9 ↔ 4x4x96:16
- Flush:543: 4x4x66:9 ↔ 4x4x96:16
- Flush:544: 4x4x66:9 ↔ 4x4x96:16
- Mate:398: 4x4x66:10 ↔ 4x4x96:7
- Flush:545: 4x4x66:10 ↔ 4x4x96:7
- Flush:546: 4x4x66:10 ↔ 4x4x96:7
- Mate:399: 4x4x66:10 ↔ 2x4x72:1
- Flush:547: 4x4x66:10 ↔ 2x4x72:1
- Flush:548: 4x4x66:4 ↔ 2x4x72:1
- Mate:400: 2x4x72:1 ↔ 2x4x88:4
- Flush:549: 2x4x72:2 ↔ 2x4x88:4
- Mate:401: 4x4x66:3 ↔ 2x4x72:2
- Mate:402: 4x4x66:4 ↔ 2x4x72:1
- Mate:403: 4x4x66:7 ↔ 2x4x120:4
- Mate:404: 2x4x48_MIR:9 ↔ leg slant_MIR:1
- Flush:550: 2x4x48_MIR:14 ↔ leg slant_MIR:1
- Mate:405: 2x4x48_MIR:14 ↔ leg slant_MIR:1
- [Mate]: 2x4x120:7 ↔ 2x4x72:11
- [Flush]: 2x4x120:7 ↔ 2x4x72:11
- [Flush]: 2x4x120:7 ↔ 2x4x72:11
- [Mate]: 2x4x120:6 ↔ 2x4x72:12
- [Flush]: 2x4x120:6 ↔ 2x4x72:12
- [Flush]: 2x4x120:6 ↔ 2x4x72:12
- [Flush]: 2x4x120:6 ↔ 2x4x88:5
- [Mate]: 2x4x120:6 ↔ 2x4x88:5
- [Flush]: 2x4x120:6 ↔ 2x4x88:5
- [Flush]: 2x4x120:6 ↔ 2x4x88:6
- [Mate]: 2x4x120:6 ↔ 2x4x88:6
- [Flush]: 2x4x120:6 ↔ 2x4x88:7
- [Mate]: 2x4x120:6 ↔ 2x4x88:7
- Mate:413: 2x4x88:5 ↔ 2x4x88:1
- Flush:561: 2x4x120:6 ↔ 2x4x120:4
- Flush:562: 2x4x88:5 ↔ 2x4x88:1
- Mate:414: 2x4x72:11 ↔ 2x4x120:5
- Flush:563: 4x4x66:8 ↔ 2x4x120:7
- Flush:564: 2x4x120:7 ↔ 2x4x120:5
- Flush:565: 2x4x120:6 ↔ back slant:1
- Flush:566: 2x4x120:6 ↔ back slant:1
- Flush:567: 2x4x120:6 ↔ back slant:1
- Mate:415: 2x4x120:7 ↔ back slant:2
- Mate:416: 2x4x120:7 ↔ back slant:2
- Flush:568: 2x4x120:7 ↔ back slant:2
- Flush:569: 2x4x88:6 ↔ 2x4x88:2
- Flush:570: 2x4x88:7 ↔ 2x4x88:3
- Mate:417: 2x4x120:7 ↔ back slant:3
- Flush:571: 2x4x72:11 ↔ back slant:3
- Mate:418: 2x4x88:7 ↔ back slant:3
- Mate:419: 2x4x120:6 ↔ back slant:4
- Flush:572: 2x4x120:6 ↔ back slant:4
- Mate:420: 2x4x88:7 ↔ back slant:4
- Flush:580: 2x4x72:12 ↔ 2x4x76:5
- Flush:581: 2x4x72:12 ↔ 2x4x76:5
- Mate:429: 2x4x72:12 ↔ 2x4x76:5
- Mate:430: 2x4x72:11 ↔ 2x4x76:6
- Flush:582: 2x4x72:11 ↔ 2x4x76:6
- Flush:583: 2x4x72:11 ↔ 2x4x76:6
- Mate:431: 2x4x120:6 ↔ 2x4x76:7
- Flush:584: 2x4x120:6 ↔ 2x4x76:7
- Mate:432 (2387.6 mm): 2x4x76:5 ↔ 2x4x76:7
- Mate:433: 2x4x120:7 ↔ 2x4x76:8
- Flush:585: 2x4x120:7 ↔ 2x4x76:8
- Mate:434 (2387.6 mm): 2x4x76:6 ↔ 2x4x76:8
- Mate:435: back slant:2 ↔ 2X4X65.191:3
- Mate:436: back slant:2 ↔ 2X4X65.191:3
- Flush:586: back slant:2 ↔ 2X4X65.191:3
- Flush:587: 2X4X65.191:3 ↔ 2x4x76:8
- Mate:437: back slant:1 ↔ 2X4X65.191:4
- Mate:438: back slant:1 ↔ 2X4X65.191:4
- Flush:588: back slant:1 ↔ 2X4X65.191:4
- Flush:589: 2x4x76:5 ↔ 2X4X92:1
- Flush:590: 2x4x76:5 ↔ 2X4X92:1
- Flush:591: 2x4x76:6 ↔ 2X4X92:2
- Mate:439: 2x4x76:6 ↔ 2X4X92:2
- Flush:592: 2x4x76:6 ↔ 2X4X92:2
- Mate:440: 2X4X92:1 ↔ 2x4x88:9
- Flush:593: 2X4X92:1 ↔ 2x4x88:9
- Flush:594: 2X4X92:1 ↔ 2x4x88:9
- Mate:441: 2X4X92:1 ↔ 2x4x88:10
- Flush:595: 2X4X65.191:4 ↔ 2x4x88:10
- Flush:596: 2x4x76:7 ↔ 2x4x88:10
- Mate:442: 2X4X65.191:3 ↔ 2X4X92:3
- Flush:597: 2X4X65.191:3 ↔ 2X4X92:3
- Mate:443: 2X4X65.191:3 ↔ 2X4X92:3
- Flush:598: back slant:4 ↔ wrapping paper:1
- Flush:599: back slant:4 ↔ wrapping paper:1
- Flush:600: 2x4x88:9 ↔ paperbodyfront:1
- Flush:601: paperbodyfront:1 ↔ 2x4x88:3
- Mate:444: 2X4X92:1 ↔ 2x4x72:15
- Flush:602: 2X4X92:1 ↔ 2x4x72:15
- Flush:603: 2X4X92:1 ↔ 2x4x72:15
- Mate:445: 2X4X92:2 ↔ 2x4x72:13
- Flush:604: 2X4X92:2 ↔ 2x4x72:13
- Flush:605: 2X4X92:2 ↔ 2x4x72:13
- Flush:606: 4x4x66:5 ↔ 2x4x88:7
- Flush:607: 2x4x76:5 ↔ 2X4X92:1
## Named parameters: sa_0 = 22241.1, d253_d234 = 0 mm, d254_d240 = 0 mm, d255_d242 = 0 mm, d256_d247 = 0 mm, d257_d248 = 0 mm, d258_d249 = 0 mm, d259_d250 = 0 mm, d260_d251 = 0 mm, d261_d252 = 0 mm, sa_1 = 980.999, d827_d499 = 0 mm, d828_d500 = 0 mm, d829_d326 = 0 mm, d830_d327 = 0 mm, d831_d305 = 0 mm, d832_d306 = 0 mm, d833_d311 = 0 mm, d834_d312 = 0 mm, d835_d313 = 0 mm, d836_d314 = 0 mm, d837_d315 = 0 mm, d838_d316 = 0 mm, d839_d317 = 0 mm, d840_d143 = 0 mm, d841_d144 = 0 mm, d842_d145 = 0 mm, d843_d146 = 0 mm, d844_d147 = 203.2 mm, d845_d148 = 203.2 mm, d846_d149 = 0 mm, d847_d150 = 0 mm, d848_d61 = 0 mm, d849_d62 = 0 mm, d850_d63 = 609.6 mm, d851_d68 = 101.6 mm, d852_d69 = 0 mm, d853_d70 = 101.6 mm, d854_d71 = 0 mm, d855_d72 = 101.6 mm, d856_d73 = 0 mm, d857_d74 = 0 mm, d858_d75 = 0 mm, d859_d76 = 0 mm, d860_d77 = 0 mm, d861_d78 = 0 mm, d862_d79 = 0 mm, d863_d80 = 0 mm, d864_d136_d47_d36 = 0 mm, d865_d137_d48_d37 = 0 mm, d866_d138_d49_d38 = 0 mm, d867_d139_d50_d39 = 0 mm, d868_d31 = 0 mm, d869_d32 = 0 mm, d870_d33 = 0 mm, d871_d34 = 0 mm, d872_d35 = 0 mm, d873_d36 = 0 mm, d874_d37 = 0 mm, d875_d38 = 0 mm, d876_d39 = 0 mm, d877_d29 = 0 mm, d878_d30 = 0 mm, d879_d626 = 0 mm, d880_d319 = 0 mm, d881_d320 = 0 mm, d882_d321 = 0 mm, d883_d322 = 0 mm, d884_d323 = 0 mm, d885_d324 = 0 mm, d886_d325 = 0 mm, d887_d299 = 0 mm, d888_d301 = 0 mm, d889_d309 = 0 mm, d890_d310 = 0 mm, d891_d318 = 0 mm, d892_d245 = 0 mm, d893_d246 = 0 mm, d894_d154_d144 = 0 mm, d895_d155_d145 = 0 mm, d896_d156_d146 = 0 mm, d897_d157_d147 = 203.2 mm, d898_d158_d148 = 203.2 mm, d899_d159_d149 = 0 mm, d900_d168_d136_d47_d36 = 0 mm, d901_d169_d137_d48_d37 = 0 mm, d902_d170_d138_d49_d38 = 0 mm, d903_d171_d139_d50_d39 = 0 mm, d904_d173_d61 = 0 mm, d905_d174_d62 = 0 mm, d906_d175_d63 = 609.6 mm, d907_d176_d68 = 101.6 mm, d908_d177_d69 = 0 mm, d909_d178_d70 = 101.6 mm, d910_d179_d71 = 0 mm, d911_d182_d74 = 0 mm, d912_d183_d75 = 0 mm, d913_d184_d76 = 0 mm, d914_d185_d77 = 0 mm, d915_d186_d78 = 0 mm, d916_d187_d79 = 0 mm, d917_d188_d80 = 0 mm, d918_d190_d31 = 0 mm, d919_d191_d32 = 0 mm, d920_d192_d33 = 0 mm, d921_d193_d34 = 0 mm, d922_d194_d35 = 0 mm, d923_d195_d36 = 0 mm, d924_d196_d37 = 0 mm, d925_d197_d38 = 0 mm, d926_d198_d39 = 0 mm, d927_d210_d29 = 0 mm, d928_d211_d30 = 0 mm, d1102_d1093 = 0 mm, d1103_d1094 = 0 mm, d1104_d1098 = 0 mm, d1105_d1099 = 0 mm, d1106_d1100 = 0 mm, d1107_d1101 = 0 mm, d1108_d1095 = 0 mm, d1109_d1096 = 0 mm, d1110_d1097 = 0 mm, d1131_d1130 = 0 mm, d1132_d1122 = 0 mm, d1133_d1123 = 0 mm, d1134_d1124 = 0 mm, d1135_d1125 = 0 mm, d1136_d1126 = 0 mm, d1137_d1127 = 0 mm, d1138_d1128 = 0 mm, d1139_d1129 = 0 mm, d1140_d1102_d1093 = 0 mm, d1141_d1103_d1094 = 0 mm, d1142_d1104_d1098 = 0 mm, d1143_d1105_d1099 = 0 mm, d1144_d1106_d1100 = 0 mm, d1145_d1107_d1101 = 0 mm, d1146_d1108_d1095 = 0 mm, d1147_d1109_d1096 = 0 mm, d1148_d1110_d1097 = 0 mm, d1161_d772_d512 = 0 mm, d1162_d773_d513 = 0 mm, d1163_d774_d514 = 0 mm, d1164_d778_d437_d327 = 0 mm, d1167_d799_d405_d149 = 0 mm, d1168_d800_d406_d150 = 0 mm, d1173_d812_d418_d76 = 0 mm, d1174_d813_d419_d77 = 0 mm, d1175_d814_d420_d78 = 0 mm, d1176_d815_d421_d79 = 0 mm, d1177_d816_d422_d80 = 0 mm, d1342_d1060 = 0 mm, d1343_d1061 = 0 mm, d1344_d1062 = 0 mm, d1345_d1063 = 0 mm, d1346_d1064 = 0 mm, d1347_d1066 = 0 mm, d1348_d1068 = 0 mm, d1351_d1036 = 0 mm, d1352_d1037 = 0 mm, d1353_d1038 = 0 mm, d1354_d1039 = 0 mm, d1355_d1040 = 0 mm, d1356_d1041 = 0 mm
note: some values were not read from the file. Shown as the stored number, unit unknown: "sa_0", "sa_1".
